# Autodesk Inventor assembly: Functioning swerve drive (shaft axel)
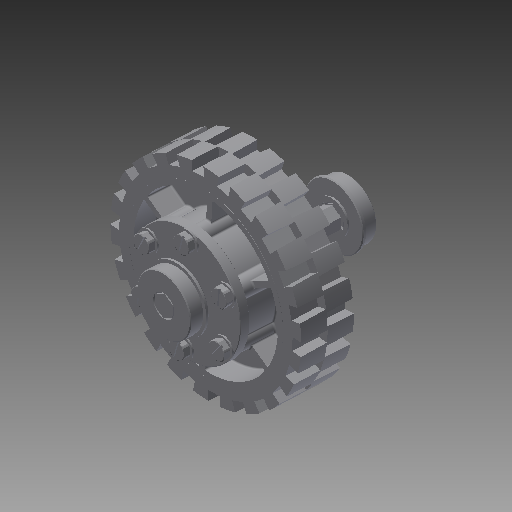
[picture p0: Inventor's stored thumbnail of the model, 512x512]
Saved by Autodesk Inventor 2019 (Build 230136000, 136)
## iProperties
Created: 2019-01-14
Part Number: Functioning swerve drive (shaft axel)
Document SubType Name: Assembly
Designer: josh
Mass: 173.357 g
Surface Area: 1034.5 cm^2
Volume: 173.357 cm^3
Density: 1 g/cm^3
Author: josh
## Documents named in this file (9)
- D:\Synthesis Robots\Epsilon\Functioning swerve drive (shaft axel).iam
- D:\Synthesis Robots\Epsilon\FR6ZZ-L Hex Bearing.ipt
- D:\Synthesis Robots\Epsilon\375 Hex Output Shaft Rev 2.ipt
- D:\Synthesis Robots\Epsilon\375 Hex Hub.ipt
- D:\Synthesis Robots\Epsilon\10-24 Hex Washer Rolling x 3-4_93882A213.ipt
- D:\Synthesis Robots\Epsilon\125x443 spacer SPS-0750-0443-0125.ipt
- D:\Synthesis Robots\Epsilon\375 E-klip - Mcm 97431A320_97431A320.ipt
- D:\Synthesis Robots\Epsilon\40t 1-25mod bevel gear.ipt
- D:\Synthesis Robots\Epsilon\4 in HiGrip Wheel.iam
## Components (14 placed, 8 different names)
1. FR6ZZ-L Hex Bearing:1
2. FR6ZZ-L Hex Bearing:2
3. 375 Hex Output Shaft Rev 2:1
4. 375 Hex Hub:1
5. 10-24 Hex Washer Rolling x 3-4_93882A213:1
6. 10-24 Hex Washer Rolling x 3-4_93882A213:2
7. 10-24 Hex Washer Rolling x 3-4_93882A213:3
8. 10-24 Hex Washer Rolling x 3-4_93882A213:4
9. 10-24 Hex Washer Rolling x 3-4_93882A213:5
10. 10-24 Hex Washer Rolling x 3-4_93882A213:6
11. 125x443 spacer SPS-0750-0443-0125:1
12. 375 E-klip - Mcm 97431A320_97431A320:1
13. 40t 1-25mod bevel gear:1
14. 4 in HiGrip Wheel:1 [sub-assembly]
## Relationships (29: Mate 28, Flush 1)
- [Mate]: 375 Hex Hub:1 ↔ 10-24 Hex Washer Rolling x 3-4_93882A213:6
- [Mate]: 375 Hex Hub:1 ↔ 10-24 Hex Washer Rolling x 3-4_93882A213:1
- [Mate]: 375 Hex Hub:1 ↔ 10-24 Hex Washer Rolling x 3-4_93882A213:5
- [Mate]: 375 Hex Hub:1 ↔ 10-24 Hex Washer Rolling x 3-4_93882A213:4
- [Mate]: 375 Hex Hub:1 ↔ 10-24 Hex Washer Rolling x 3-4_93882A213:3
- [Mate]: 375 Hex Hub:1 ↔ 10-24 Hex Washer Rolling x 3-4_93882A213:2
- [Mate]: 375 Hex Hub:1 ↔ 10-24 Hex Washer Rolling x 3-4_93882A213:2
- [Mate]: 375 Hex Hub:1 ↔ 10-24 Hex Washer Rolling x 3-4_93882A213:4
- [Mate]: 375 Hex Hub:1 ↔ 10-24 Hex Washer Rolling x 3-4_93882A213:3
- [Mate]: 375 Hex Hub:1 ↔ 10-24 Hex Washer Rolling x 3-4_93882A213:1
- [Mate]: 375 Hex Hub:1 ↔ 10-24 Hex Washer Rolling x 3-4_93882A213:6
- [Mate]: 375 Hex Hub:1 ↔ 10-24 Hex Washer Rolling x 3-4_93882A213:5
- [Mate]: 375 Hex Output Shaft Rev 2:1 ↔ 375 Hex Hub:1
- [Mate]: 375 Hex Output Shaft Rev 2:1 ↔ 375 Hex Hub:1
- [Mate]: FR6ZZ-L Hex Bearing:1 ↔ 375 Hex Output Shaft Rev 2:1
- [Mate]: FR6ZZ-L Hex Bearing:1 ↔ 375 Hex Output Shaft Rev 2:1
- [Mate]: 375 Hex Output Shaft Rev 2:1 ↔ 40t 1-25mod bevel gear:1
- [Mate]: 375 Hex Output Shaft Rev 2:1 ↔ 40t 1-25mod bevel gear:1
- [Mate]: FR6ZZ-L Hex Bearing:1 ↔ 125x443 spacer SPS-0750-0443-0125:1
- [Mate]: FR6ZZ-L Hex Bearing:1 ↔ 125x443 spacer SPS-0750-0443-0125:1
- [Mate]: 375 Hex Output Shaft Rev 2:1 ↔ 375 E-klip - Mcm 97431A320_97431A320:1
- [Mate]: 375 Hex Output Shaft Rev 2:1 ↔ 375 E-klip - Mcm 97431A320_97431A320:1
- [Mate]: 375 Hex Hub:1 ↔ 125x443 spacer SPS-0750-0443-0125:1
- [Flush]: FR6ZZ-L Hex Bearing:1 ↔ 375 Hex Output Shaft Rev 2:1
- [Mate]: 10-24 Hex Washer Rolling x 3-4_93882A213:6 ↔ 4 in HiGrip Wheel:1
- [Mate]: 10-24 Hex Washer Rolling x 3-4_93882A213:5 ↔ 4 in HiGrip Wheel:1
- [Mate]: 10-24 Hex Washer Rolling x 3-4_93882A213:4 ↔ 4 in HiGrip Wheel:1
- [Mate]: 375 Hex Hub:1 ↔ 4 in HiGrip Wheel:1
- [Mate]: 40t 1-25mod bevel gear:1 ↔ 4 in HiGrip Wheel:1
## Named parameters: d310_d102 = 0 mm, d311_d103 = 0 mm, d312_d104 = 0 mm, d313_d105 = 0 mm, d314_d106 = 0 mm, d315_d107 = 0 mm, d316_d108 = 0 mm, d317_d109 = 0 mm, d318_d110 = 0 mm, d319_d113 = 0 mm, d320_d114 = 0 mm, d325_d121 = 0 mm, d326_d122 = 0 mm, d327_d131 = 0 mm, d328_d132 = 0 mm, d329_d135 = 0 mm, d330_d136 = 0 mm, d333_d95 = 0 mm, d334_d96 = 0 mm, d335_d97 = 0 mm, d336_d98 = 0 mm, d337_d99 = 0 mm, d338_d100 = 0 mm, d339_d101 = 0 mm, d341_d126 = 0 mm, d342_d127 = 0 mm, d343_d128 = 0 mm, d344_d129 = 0 mm, d345_d162 = 0 mm
